# Autodesk Inventor assembly: ExteriorBumperCar2
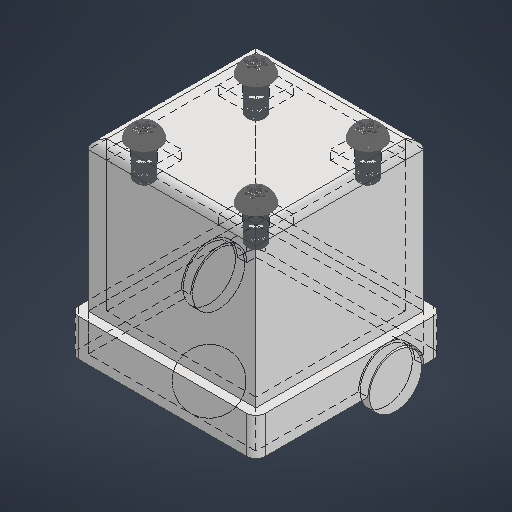
[picture p0: Inventor's stored thumbnail of the model, 512x512]
Saved by Autodesk Inventor 2026.1 (Build 301233000, 233)
## iProperties
Created: 2026-06-28
Part Number: ExteriorBumperCar2
Document SubType Name: Assembly
Designer: Kasi Pusuluri
Author: Kasi Pusuluri
## Documents named in this file (7)
- C:\Users\Kasi Pusuluri\Documents\Outpost 2026\BumperCarV2\ExteriorBumperCar2.iam
- C:\Users\Kasi Pusuluri\Documents\Outpost 2026\BumperCarV2\Top1.ipt
- C:\Users\Kasi Pusuluri\Documents\Outpost 2026\BumperCarV2\BumperBody.ipt
- C:\Users\Kasi Pusuluri\Documents\Outpost 2026\BumperCarV2\Connector1.ipt
- C:\Users\Kasi Pusuluri\Downloads\EDLG-J2D4-M6-L12.ipt
- C:\Users\Kasi Pusuluri\Documents\Outpost 2026\BumperCarV2\BumperWheel.ipt
- C:\Users\Kasi Pusuluri\Documents\Outpost 2026\BumperCarV2\BumperCaster.ipt
## Components (13 placed, 6 different names)
1. BumperBody:1 — Mate:1, Mate:2
2. Top1:1 — Rotational:1, Rotational:2, Rotational:3, Rotational:4, Rotational:5, Rotational:6, Rotational:7, Rotational:8, Mate:1, Mate:2
3. Connector1:1 — Rotational:2
4. Connector1:2 — Rotational:1
5. Connector1:3 — Rotational:4
6. Connector1:4 — Rotational:3
7. EDLG-J2D4-M6-L12:1 — Rotational:8
8. EDLG-J2D4-M6-L12:2 — Rotational:7
9. EDLG-J2D4-M6-L12:3 — Rotational:6
10. EDLG-J2D4-M6-L12:4 — Rotational:5
11. BumperWheel:1
12. BumperWheel:2
13. BumperCaster:1
## Relationships (10: RevoluteJoint 8, Mate 2)
- Rotational:1 [RevoluteJoint]: Top1:1 ↔ Connector1:2
- Rotational:2 [RevoluteJoint]: Top1:1 ↔ Connector1:1
- Rotational:3 [RevoluteJoint]: Top1:1 ↔ Connector1:4
- Rotational:4 [RevoluteJoint]: Top1:1 ↔ Connector1:3
- Rotational:5 [RevoluteJoint]: Top1:1 ↔ EDLG-J2D4-M6-L12:4
- Rotational:6 [RevoluteJoint]: Top1:1 ↔ EDLG-J2D4-M6-L12:3
- Rotational:7 [RevoluteJoint]: Top1:1 ↔ EDLG-J2D4-M6-L12:2
- Rotational:8 [RevoluteJoint]: Top1:1 ↔ EDLG-J2D4-M6-L12:1
- Mate:1: BumperBody:1 ↔ Top1:1
- Mate:2: BumperBody:1 ↔ Top1:1
